# Autodesk Inventor assembly: two-section-bellows-on-bearings
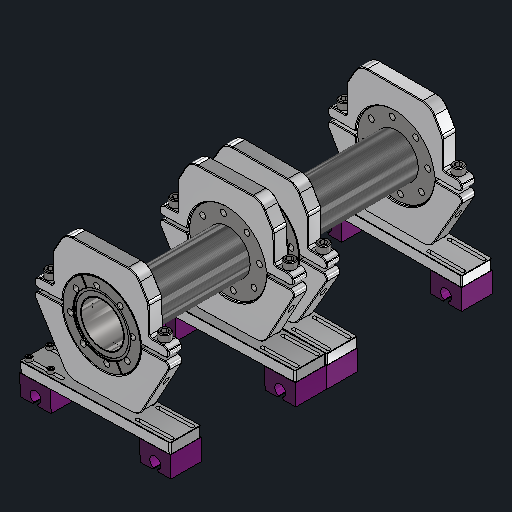
[picture p0: Inventor's stored thumbnail of the model, 512x512]
Saved by Autodesk Inventor 2027.1 (Build 311270010, 270A)
## iProperties
Part Number: two-section-bellows-on-bearings
Document SubType Name: Assembly
Designer: queezz
Author: queezz
## Documents named in this file (8)
- C:\Users\queezz\Dropbox\Drawings\pihti-cad\bellows-probe\two-section-bellows-on-bearings.iam
- C:\Users\queezz\Dropbox\Drawings\pihti-cad\bellows-probe\flange-camp-114.ipt
- C:\Users\queezz\Dropbox\Drawings\pihti-cad\bellows-probe\bellows_flange.ipt
- C:\Users\queezz\Dropbox\Drawings\pihti-cad\bellows-probe\linearbearing.ipt
- C:\Users\queezz\Dropbox\Drawings\pihti-cad\bellows-probe\instead-of-bellows.ipt
- C:\Users\queezz\Dropbox\Drawings\pihti-cad\bellows-probe\clamp-foot.ipt
- C:\Users\queezz\Documents\Inventor\Content Center Files\R2027\en-US\AS 1420\AS 1420 - 1973 - M10 x 30.ipt
- C:\Users\queezz\Dropbox\Drawings\pihti-cad\ContentCenter\Fastners\M5x20-SHCS.ipt
## Components (42 placed, 7 different names)
1. flange-camp-114:1
2. flange-camp-114:2
3. bellows_flange:1
4. bellows_flange:2
5. linearbearing:1
6. linearbearing:2
7. linearbearing:3
8. linearbearing:4
9. instead-of-bellows:1
10. instead-of-bellows:2
11. clamp-foot:1
12. clamp-foot:2
13. instead-of-bellows:3
14. instead-of-bellows:4
15. AS 1420 - Metric M10 x 30:1
16. AS 1420 - Metric M10 x 30:2
17. AS 1420 - Metric M10 x 30:3
18. AS 1420 - Metric M10 x 30:4
19. AS 1420 - Metric M5 x 20:1
20. AS 1420 - Metric M5 x 20:2
21. AS 1420 - Metric M5 x 20:3
22. flange-camp-114:3
23. flange-camp-114:4
24. bellows_flange:3
25. bellows_flange:4
26. linearbearing:5
27. linearbearing:6
28. linearbearing:7
29. linearbearing:8
30. instead-of-bellows:5
31. instead-of-bellows:6
32. clamp-foot:3
33. clamp-foot:4
34. instead-of-bellows:7
35. instead-of-bellows:8
36. AS 1420 - Metric M10 x 30:5
37. AS 1420 - Metric M10 x 30:6
38. AS 1420 - Metric M10 x 30:7
39. AS 1420 - Metric M10 x 30:8
40. AS 1420 - Metric M5 x 20:4
41. AS 1420 - Metric M5 x 20:5
42. AS 1420 - Metric M5 x 20:6
## Relationships (90: Mate 34, Flush 30, WeldJoint 20, Angle 4, RevoluteJoint 2)
- [Mate]: clamp-foot:1 ↔ clamp-foot:4
- [Mate]: linearbearing:1 ↔ linearbearing:8
- [Flush]: flange-camp-114:1 ↔ clamp-foot:2
- [Mate]: flange-camp-114:1 ↔ clamp-foot:2
- [Mate]: flange-camp-114:1 ↔ clamp-foot:2
- [WeldJoint]: flange-camp-114:1 ↔ bellows_flange:2
- [WeldJoint]: flange-camp-114:1 ↔ AS 1420 - Metric M10 x 30:2
- [WeldJoint]: flange-camp-114:1 ↔ AS 1420 - Metric M10 x 30:1
- [Flush]: flange-camp-114:1 ↔ bellows_flange:2
- [Mate]: flange-camp-114:1 ↔ bellows_flange:2
- [Angle] (150 deg): flange-camp-114:1 ↔ bellows_flange:2
- [Mate]: flange-camp-114:2 ↔ clamp-foot:1
- [Mate]: flange-camp-114:2 ↔ clamp-foot:1
- [Flush]: flange-camp-114:2 ↔ clamp-foot:1
- [WeldJoint]: flange-camp-114:2 ↔ bellows_flange:1
- [WeldJoint]: flange-camp-114:2 ↔ AS 1420 - Metric M10 x 30:4
- [WeldJoint]: flange-camp-114:2 ↔ AS 1420 - Metric M10 x 30:3
- [Flush]: flange-camp-114:2 ↔ bellows_flange:1
- [Mate]: flange-camp-114:2 ↔ bellows_flange:1
- [Angle] (30 deg): flange-camp-114:2 ↔ bellows_flange:1
- [WeldJoint]: bellows_flange:1 ↔ instead-of-bellows:2
- [Mate] (-650 mm): bellows_flange:1 ↔ bellows_flange:2
- [WeldJoint]: bellows_flange:2 ↔ instead-of-bellows:1
- [Flush]: linearbearing:1 ↔ linearbearing:3
- [Flush]: linearbearing:1 ↔ clamp-foot:1
- [Mate]: linearbearing:1 ↔ linearbearing:4
- [Flush]: linearbearing:1 ↔ clamp-foot:1
- [Flush]: linearbearing:2 ↔ linearbearing:4
- [Flush]: linearbearing:2 ↔ linearbearing:4
- [Mate]: linearbearing:2 ↔ linearbearing:3
- [Flush]: linearbearing:2 ↔ clamp-foot:2
- [Mate]: linearbearing:3 ↔ clamp-foot:1
- [Flush]: linearbearing:3 ↔ clamp-foot:1
- [Flush]: linearbearing:3 ↔ clamp-foot:1
- [WeldJoint] (15 mm): linearbearing:3 ↔ AS 1420 - Metric M5 x 20:3
- [WeldJoint] (15 mm): linearbearing:3 ↔ AS 1420 - Metric M5 x 20:2
- [RevoluteJoint] (15 mm): linearbearing:3 ↔ AS 1420 - Metric M5 x 20:1
- [Flush]: linearbearing:4 ↔ clamp-foot:2
- [Flush]: linearbearing:4 ↔ clamp-foot:2
- [Flush]: linearbearing:4 ↔ clamp-foot:2
- [Mate]: instead-of-bellows:1 ↔ instead-of-bellows:2
- [Mate]: instead-of-bellows:1 ↔ instead-of-bellows:4
- [Mate] (-200 mm): instead-of-bellows:1 ↔ instead-of-bellows:4
- [Mate]: instead-of-bellows:2 ↔ instead-of-bellows:3
- [Mate]: instead-of-bellows:2 ↔ instead-of-bellows:3
- [Mate]: instead-of-bellows:3 ↔ instead-of-bellows:4
- [Flush]: flange-camp-114:3 ↔ clamp-foot:4
- [Mate]: flange-camp-114:3 ↔ clamp-foot:4
- [Mate]: flange-camp-114:3 ↔ clamp-foot:4
- [WeldJoint]: flange-camp-114:3 ↔ bellows_flange:4
- [WeldJoint]: flange-camp-114:3 ↔ AS 1420 - Metric M10 x 30:6
- [WeldJoint]: flange-camp-114:3 ↔ AS 1420 - Metric M10 x 30:5
- [Flush]: flange-camp-114:3 ↔ bellows_flange:4
- [Mate]: flange-camp-114:3 ↔ bellows_flange:4
- [Angle] (150 deg): flange-camp-114:3 ↔ bellows_flange:4
- [Mate]: flange-camp-114:4 ↔ clamp-foot:3
- [Mate]: flange-camp-114:4 ↔ clamp-foot:3
- [Flush]: flange-camp-114:4 ↔ clamp-foot:3
- [WeldJoint]: flange-camp-114:4 ↔ bellows_flange:3
- [WeldJoint]: flange-camp-114:4 ↔ AS 1420 - Metric M10 x 30:8
- [WeldJoint]: flange-camp-114:4 ↔ AS 1420 - Metric M10 x 30:7
- [Flush]: flange-camp-114:4 ↔ bellows_flange:3
- [Mate]: flange-camp-114:4 ↔ bellows_flange:3
- [Angle] (30 deg): flange-camp-114:4 ↔ bellows_flange:3
- [WeldJoint]: bellows_flange:3 ↔ instead-of-bellows:6
- [Mate] (-650 mm): bellows_flange:3 ↔ bellows_flange:4
- [WeldJoint]: bellows_flange:4 ↔ instead-of-bellows:5
- [Flush]: linearbearing:5 ↔ linearbearing:7
- [Flush]: linearbearing:5 ↔ clamp-foot:3
- [Mate]: linearbearing:5 ↔ linearbearing:8
- [Flush]: linearbearing:5 ↔ clamp-foot:3
- [Flush]: linearbearing:6 ↔ linearbearing:8
- [Flush]: linearbearing:6 ↔ linearbearing:8
- [Mate]: linearbearing:6 ↔ linearbearing:7
- [Flush]: linearbearing:6 ↔ clamp-foot:4
- [Mate]: linearbearing:7 ↔ clamp-foot:3
- [Flush]: linearbearing:7 ↔ clamp-foot:3
- [Flush]: linearbearing:7 ↔ clamp-foot:3
- [WeldJoint] (15 mm): linearbearing:7 ↔ AS 1420 - Metric M5 x 20:6
- [WeldJoint] (15 mm): linearbearing:7 ↔ AS 1420 - Metric M5 x 20:5
- [RevoluteJoint] (15 mm): linearbearing:7 ↔ AS 1420 - Metric M5 x 20:4
- [Flush]: linearbearing:8 ↔ clamp-foot:4
- [Flush]: linearbearing:8 ↔ clamp-foot:4
- [Flush]: linearbearing:8 ↔ clamp-foot:4
- [Mate]: instead-of-bellows:5 ↔ instead-of-bellows:6
- [Mate]: instead-of-bellows:5 ↔ instead-of-bellows:8
- [Mate] (-200 mm): instead-of-bellows:5 ↔ instead-of-bellows:8
- [Mate]: instead-of-bellows:6 ↔ instead-of-bellows:7
- [Mate]: instead-of-bellows:6 ↔ instead-of-bellows:7
- [Mate]: instead-of-bellows:7 ↔ instead-of-bellows:8
## Named parameters: d35_d44 = 0 mm, d24_d26 = 0 mm, d53_d56 = 0 mm, d78_d39 = 0 mm, d79_d113 = 0 mm, d80_d114 = 0 mm, d81_d55 = 0 mm, d82_d67 = 0 mm, d83_d68 = 150 deg, d84_d109 = 0 mm, d85_d33 = 0 mm, d86_d34 = 0 mm, d87_d111 = 0 mm, d88_d112 = 0 mm, d89_d69 = 0 mm, d90_d70 = 0 mm, d95_d75 = 30 deg, d96_d110 = 0 mm, d98_d71 = 0 mm, d99_d72 = 0 mm, d100_d73 = 0 mm, d101_d40 = -650 mm, d102_d41 = -135 mm, d103_d42 = -485 mm, d104_d22 = 0 mm, d105_d21 = 0 mm, d106_d36 = 0 mm, d107_d45 = 0 mm, d108_d74 = 0 mm, d115_d18 = 0 mm, d116_d37 = 0 mm, d117_d43 = 0 mm, d118_d17 = 0 mm, d119_d19 = 0 mm, d121_d97 = 15 mm, d122_d92 = 15 mm, d123_d93 = 15 mm, d124_d94 = -1.444006 deg, d126_d91 = 0 mm, d127_d24_d26 = 0 mm, d128_d35 = 0 mm, d129_d38 = 0 mm, d130_d46 = 0 mm, d132_d61 = -200 mm, d133_d62 = 0 mm, d134_d63 = -200 mm, d135_d23 = 0 mm, d136_d57 = 0 mm, d137_d58 = 0 mm, d138_d59 = 0 mm, d139_d60 = -200 mm, d140_d64 = 0 mm, d141_d65 = 0 mm, d142_d66 = -200 mm
